# Autodesk Inventor assembly: Actuator 1.5
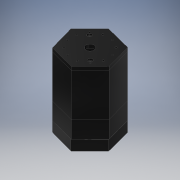
[picture p0: Inventor's stored thumbnail of the model, 180x180]
Saved by Autodesk Inventor 2017 SP1 (Build 210196100, 196)
## iProperties
Created: 2019-08-28
Part Number: Actuator 1.5
Document SubType Name: Assembly
Designer: Dell
Author: Dell
## Documents named in this file (12)
- C:\Users\Zach\Documents\GitHub\tr2\Actuator 1.5\Actuator 1.5.iam
- C:\Users\Zach\Documents\GitHub\tr2\Actuator 1.5\Slewing.iam
- C:\Users\Zach\Documents\GitHub\tr2\Actuator 1.5\AC01.ipt
- C:\Users\Zach\Documents\GitHub\tr2\Actuator 1.5\AC02.ipt
- C:\Users\Zach\Documents\GitHub\tr2\Actuator 1.5\12RPM Gear Motor.ipt
- C:\Users\Zach\Documents\GitHub\tr2\Actuator 1.5\AC03.ipt
- C:\Users\Zach\Documents\GitHub\tr2\Actuator 1.5\AEAT-6012.ipt
- C:\Users\Zach\Documents\GitHub\tr2\Actuator 1.5\AC04.ipt
- C:\Users\Zach\Documents\GitHub\tr2\Actuator 1.5\SEA Gearbox.iam
- C:\Users\Zach\Documents\GitHub\tr2\Actuator 1.5\AC05.ipt
- C:\Users\Zach\slaterobots.com\Slate Robotics OneDrive - Documents\CodyM\QTC_KSS1_5-12A.ipt
- C:\Users\Zach\Documents\GitHub\tr2\Actuator 1.5\SEA Gearbox\Design Accelerator\Spur Gears3.iam
## Components (13 placed, 11 different names)
1. Slewing:1 [sub-assembly] — Mate:3, Mate:4, Mate:56, Mate:57, Mate:58, Mate:59
2. AC01:1 — Mate:3, Mate:4, Mate:23, Mate:35, Mate:50, Mate:59
3. AC02:1 — Mate:13, Mate:14, Mate:23, Mate:34, Mate:35, Mate:38, Mate:39, Mate:42, Mate:45, Mate:46, Mate:55, Mate:60, Mate:62, Mate:63, Mate:64, Mate:66
4. AC03:1
5. AC04:1 — Mate:42, Mate:45, Mate:46
6. AC05:1 — Mate:56, Mate:57
7. 12RPM Gear Motor:1 — Mate:13, Mate:14, Mate:34, Mate:61
8. AEAT-6012:1 — Mate:38, Mate:39, Mate:60, Mate:68
9. SEA Gearbox:1 [sub-assembly] — Mate:50, Mate:55, Mate:58, Mate:67, Mate:69
10. QTC_KSS1_5-12A:1 — Mate:61, Mate:67
11. AEAT-6012:2 — Mate:62, Mate:63, Mate:64, Mate:65
12. Spur Gears:6 [sub-assembly] — Mate:65, Mate:66
13. QTC_KSS1_5-12A:2 — Mate:68, Mate:69
## Relationships (28: Mate 28)
- Mate:3: Slewing:1 ↔ AC01:1
- Mate:4: Slewing:1 ↔ AC01:1
- Mate:13: AC02:1 ↔ 12RPM Gear Motor:1
- Mate:14: AC02:1 ↔ 12RPM Gear Motor:1
- Mate:23: AC01:1 ↔ AC02:1
- Mate:34: AC02:1 ↔ 12RPM Gear Motor:1
- Mate:35: AC01:1 ↔ AC02:1
- Mate:38: AC02:1 ↔ AEAT-6012:1
- Mate:39: AC02:1 ↔ AEAT-6012:1
- Mate:42: AC02:1 ↔ AC04:1
- Mate:45: AC02:1 ↔ AC04:1
- Mate:46: AC02:1 ↔ AC04:1
- Mate:50: AC01:1 ↔ SEA Gearbox:1
- Mate:55: AC02:1 ↔ SEA Gearbox:1
- Mate:56: Slewing:1 ↔ AC05:1
- Mate:57: Slewing:1 ↔ AC05:1
- Mate:58: Slewing:1 ↔ SEA Gearbox:1
- Mate:59: Slewing:1 ↔ AC01:1
- Mate:60: AC02:1 ↔ AEAT-6012:1
- Mate:61: 12RPM Gear Motor:1 ↔ QTC_KSS1_5-12A:1
- Mate:62: AC02:1 ↔ AEAT-6012:2
- Mate:63: AC02:1 ↔ AEAT-6012:2
- Mate:64: AC02:1 ↔ AEAT-6012:2
- Mate:65: AEAT-6012:2 ↔ Spur Gears:6
- Mate:66: AC02:1 ↔ Spur Gears:6
- Mate:67: SEA Gearbox:1 ↔ QTC_KSS1_5-12A:1
- Mate:68: AEAT-6012:1 ↔ QTC_KSS1_5-12A:2
- Mate:69: SEA Gearbox:1 ↔ QTC_KSS1_5-12A:2
